# Autodesk Inventor assembly: wahacz_zewn_zlozenie
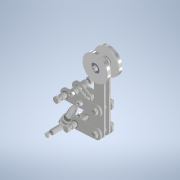
[picture p0: Inventor's stored thumbnail of the model, 180x180]
Saved by Autodesk Inventor 2020.3 (Build 243373000, 373)
## iProperties
Created: 2021-10-24
Part Number: wahacz_zewn_zlozenie
Document SubType Name: Assembly
Designer: patry
Author: patry
## Documents named in this file (26)
- C:\Users\patry\Desktop\Semestr 7\Inzynierka\Projekt inventor\Ariadna_inzynierka\Workspaces\Obszar roboczy\Obszar roboczy\Naped\Zawieszenie_v3\wahacz_zewn_zlozenie.iam
- C:\Users\patry\Desktop\Semestr 7\Inzynierka\Projekt inventor\Ariadna_inzynierka\Workspaces\Obszar roboczy\Obszar roboczy\Naped\Zawieszenie_v3\ramie_1_wahacza.ipt
- C:\Users\patry\Desktop\Semestr 7\Inzynierka\Projekt inventor\Ariadna_inzynierka\Workspaces\Obszar roboczy\Obszar roboczy\Naped\Zawieszenie_v3\ramie_2_wahacza.ipt
- C:\Users\patry\Desktop\Semestr 7\Inzynierka\Projekt inventor\Ariadna_inzynierka\Workspaces\Obszar roboczy\Obszar roboczy\Naped\Zawieszenie_v3\tuleja_TUF106040.ipt
- C:\Users\patry\Desktop\Semestr 7\Inzynierka\Projekt inventor\Ariadna_inzynierka\Workspaces\Obszar roboczy\Obszar roboczy\Naped\Sruby\M6_nut_5mm.ipt
- C:\Users\patry\Desktop\Semestr 7\Inzynierka\Projekt inventor\Ariadna_inzynierka\Workspaces\Obszar roboczy\Obszar roboczy\Naped\Amortyzator\Korpus.ipt
- C:\Users\patry\Desktop\Semestr 7\Inzynierka\Projekt inventor\Ariadna_inzynierka\Workspaces\Obszar roboczy\Obszar roboczy\Naped\Amortyzator\Tlok.ipt
- C:\Users\patry\Desktop\Semestr 7\Inzynierka\Projekt inventor\Ariadna_inzynierka\Workspaces\Obszar roboczy\Obszar roboczy\Naped\Amortyzator\Nakretka.ipt
- C:\Users\patry\Desktop\Semestr 7\Inzynierka\Projekt inventor\Ariadna_inzynierka\Workspaces\Obszar roboczy\Obszar roboczy\Naped\Sruby\M5_nut_5mm.ipt
- C:\Users\patry\Desktop\Semestr 7\Inzynierka\Projekt inventor\Ariadna_inzynierka\Workspaces\Obszar roboczy\Obszar roboczy\Naped\Sruby\M5_70_shaft.ipt
- C:\Users\patry\Desktop\Semestr 7\Inzynierka\Projekt inventor\Ariadna_inzynierka\Workspaces\Obszar roboczy\Obszar roboczy\Naped\Sruby\M3_16_shaft.ipt
- C:\Users\patry\Desktop\Semestr 7\Inzynierka\Projekt inventor\Ariadna_inzynierka\Workspaces\Obszar roboczy\Obszar roboczy\Naped\Sruby\M3_nut_2,5mm.ipt
- C:\Users\patry\Desktop\Semestr 7\Inzynierka\Projekt inventor\Ariadna_inzynierka\Workspaces\Obszar roboczy\Obszar roboczy\Naped\Zawieszenie_v3\wspornik_amortyzatora.ipt
- C:\Users\patry\Desktop\Semestr 7\Inzynierka\Projekt inventor\Ariadna_inzynierka\Workspaces\Obszar roboczy\Obszar roboczy\Naped\Sruby\M6_40_shaft.ipt
- C:\Users\patry\Desktop\Semestr 7\Inzynierka\Projekt inventor\Ariadna_inzynierka\Workspaces\Obszar roboczy\Obszar roboczy\Naped\Sruby\tuleja_M6_M10_7.ipt
- C:\Users\patry\Desktop\Semestr 7\Inzynierka\Projekt inventor\Ariadna_inzynierka\Workspaces\Obszar roboczy\Obszar roboczy\Naped\Sruby\M6_1,25_pad.ipt
- C:\Users\patry\Desktop\Semestr 7\Inzynierka\Projekt inventor\Ariadna_inzynierka\Workspaces\Obszar roboczy\Obszar roboczy\Naped\Sruby\M6_70_shaft.ipt
- C:\Users\patry\Desktop\Semestr 7\Inzynierka\Projekt inventor\Ariadna_inzynierka\Workspaces\Obszar roboczy\Obszar roboczy\Naped\Sruby\M5_40_shaft.ipt
- M5_shaft.ipt
- C:\Users\patry\Desktop\Semestr 7\Inzynierka\Projekt inventor\Ariadna_inzynierka\Workspaces\Obszar roboczy\Obszar roboczy\Naped\Sruby\tuleja_M5_M9_20.ipt
- C:\Users\patry\Desktop\Semestr 7\Inzynierka\Projekt inventor\Ariadna_inzynierka\Workspaces\Obszar roboczy\Obszar roboczy\Naped\Sruby\tuleja_M5_M9_25.ipt
- C:\Users\patry\Desktop\Semestr 7\Inzynierka\Projekt inventor\Ariadna_inzynierka\Workspaces\Obszar roboczy\Obszar roboczy\Naped\Sruby\tuleja_M5_M9_4,5.ipt
- C:\Users\patry\Desktop\Semestr 7\Inzynierka\Projekt inventor\Ariadna_inzynierka\Workspaces\Obszar roboczy\Obszar roboczy\Naped\Zawieszenie_v3\glowny_wahacz_zewn.ipt
- C:\Users\patry\Desktop\Semestr 7\Inzynierka\Projekt inventor\Ariadna_inzynierka\Workspaces\Obszar roboczy\Obszar roboczy\Naped\Sruby\tuleja_M6_M10_8,5.ipt
- C:\Users\patry\Desktop\Semestr 7\Inzynierka\Projekt inventor\Ariadna_inzynierka\Workspaces\Obszar roboczy\Obszar roboczy\Naped\Sruby\tuleja_M6_M10_13,5.ipt
- C:\Users\patry\Desktop\Semestr 7\Inzynierka\Projekt inventor\Ariadna_inzynierka\Workspaces\Obszar roboczy\Obszar roboczy\Naped\Zawieszenie_v3\independent_wheel_pair.iam
## Components (65 placed, 24 different names)
1. ramie_1_wahacza:1 — Zestawiające:7, Zestawiające:8, Kątowe:4, Zestawiające:108, Zestawiające:109, Zestawiające:110, Równoległe:6, Zestawiające:114, Zestawiające:158, Równoległe:11, Zestawiające:159, Równoległe:12, Zestawiające:161, Zestawiające:163, Zestawiające:175, Zestawiające:179, Zestawiające:203, Zestawiające:204
2. ramie_2_wahacza:1 — Zestawiające:1, Zestawiające:2, Kątowe:1, Zestawiające:118, Zestawiające:206, Zestawiające:207
3. tuleja_TUF106040:1 — Zestawiające:1, Zestawiające:2, Kątowe:1, Zestawiające:93, Zestawiające:200
4. tuleja_TUF106040:2 — Zestawiające:205, Zestawiające:206, Zestawiające:207, Zestawiające:217
5. tuleja_TUF106040:3 — Zestawiające:202, Zestawiające:203, Zestawiające:204, Zestawiające:219
6. tuleja_TUF106040:4 — Zestawiające:7, Zestawiające:8, Kątowe:4, Zestawiające:111, Zestawiające:132
7. tuleja_TUF106040:5 — Zestawiające:89, Zestawiające:201, Zestawiające:216
8. tuleja_TUF106040:6 — Zestawiające:88, Zestawiające:90, Zestawiające:189, Zestawiające:198
9. ramie_2_wahacza:2 — Równoległe:7, Zestawiające:120, Zestawiające:209, Zestawiające:210
10. tuleja_TUF106040:7 — Zestawiające:93, Zestawiające:112, Zestawiające:140
11. tuleja_TUF106040:8 — Zestawiające:208, Zestawiające:209, Zestawiające:210, Zestawiające:212
12. M6_nut_5mm:2 — Zestawiające:113, Zestawiające:114
13. Korpus:1 — Walcowe:1, Zestawiające:83, Równoległe:4, Zestawiające:87, Zestawiające:169, Zestawiające:171
14. Tlok:1 — Walcowe:1, Zestawiające:102, Zestawiające:103
15. Nakretka:1
16. M5_nut_5mm:1 — Zestawiające:84, Zestawiające:86, Zestawiające:87, Równoległe:9, Równoległe:10
17. M5_70_shaft:1 — Zestawiające:83, Równoległe:4, Zestawiające:84, Zestawiające:85, Zestawiające:143, Równoległe:8, Zestawiające:168, Zestawiające:170
18. ramie_1_wahacza:3 — Zestawiające:88, Zestawiające:89, Zestawiające:90, Zestawiające:116, Zestawiające:165, Zestawiające:167, Zestawiające:173, Zestawiające:177, Zestawiające:201
19. M5_nut_5mm:2 — Zestawiające:85, Zestawiające:86
20. M3_16_shaft:1 — Zestawiające:97, Równoległe:5, Zestawiające:98, Zestawiające:100, Zestawiające:102
21. M3_nut_2,5mm:1 — Zestawiające:98, Zestawiające:99
22. M3_nut_2,5mm:2 — Zestawiające:100, Zestawiające:101
23. wspornik_amortyzatora:1 — Zestawiające:94, Zestawiające:95, Zestawiające:96, Równoległe:5, Zestawiające:99, Zestawiające:108, Zestawiające:109, Zestawiające:110
24. wspornik_amortyzatora:2 — Zestawiające:94, Zestawiające:95, Zestawiające:96, Zestawiające:97, Zestawiające:101, Zestawiające:103
25. M6_40_shaft:1 — Zestawiające:111, Równoległe:6, Zestawiające:113, Zestawiające:115, Zestawiające:121, Zestawiające:127, Zestawiające:131, Zestawiające:182, Zestawiające:186, Zestawiające:189
26. M6_40_shaft:2 — Zestawiające:112, Równoległe:7, Zestawiające:117, Zestawiające:119, Zestawiające:123, Zestawiające:135, Zestawiające:139, Zestawiające:180, Zestawiające:185
27. M6_nut_5mm:11 — Zestawiające:115, Zestawiające:116
28. M6_nut_5mm:12 — Zestawiające:117, Zestawiające:118
29. M6_nut_5mm:13 — Zestawiające:119, Zestawiające:120
30. tuleja_M6_M10_7:1 — Zestawiające:121, Zestawiające:196
31. tuleja_M6_M10_7:2 — Zestawiające:123, Zestawiające:181
32. M6_1,25_pad:1 — Zestawiające:125, Zestawiające:126, Zestawiające:127, Zestawiające:197
33. M6_1,25_pad:2 — Zestawiające:125, Zestawiające:126, Zestawiające:198
34. M6_1,25_pad:3 — Zestawiające:131, Zestawiające:132
35. M6_1,25_pad:4 — Zestawiające:194
36. M6_1,25_pad:5 — Zestawiające:135, Zestawiające:199
37. M6_1,25_pad:6 — Zestawiające:200
38. M6_1,25_pad:7 — Zestawiające:139, Zestawiające:140
39. M6_1,25_pad:8 — Zestawiające:195
40. M6_70_shaft:1 — Zestawiające:143, Zestawiające:149, Zestawiające:205, Zestawiające:208, Zestawiające:211, Zestawiające:213
41. M6_70_shaft:2 — Równoległe:8, Zestawiające:144, Zestawiające:145, Zestawiające:202, Zestawiające:215, Zestawiające:218
42. M6_nut_5mm:14 — Zestawiające:144, Zestawiające:146
43. M6_nut_5mm:15 — Zestawiające:145, Zestawiające:146, Równoległe:9
44. M6_nut_5mm:16 — Zestawiające:148, Zestawiające:149
45. M6_nut_5mm:17 — Zestawiające:148, Równoległe:10
46. M5_shaft:1 — Zestawiające:158, Równoległe:11, Zestawiające:162, Zestawiające:164, Zestawiające:172, Zestawiające:174
47. M5_shaft:2 — Zestawiające:159, Równoległe:12, Zestawiające:160, Zestawiające:166, Zestawiające:176, Zestawiające:178
48. M5_nut_5mm:3 — Zestawiające:160, Zestawiające:161
49. M5_nut_5mm:4 — Zestawiające:162, Zestawiające:163
50. M5_nut_5mm:5 — Zestawiające:164, Zestawiające:165
51. M5_nut_5mm:6 — Zestawiające:166, Zestawiające:167
52. tuleja_M5_M9_20:1 — Zestawiające:168, Zestawiające:169
53. tuleja_M5_M9_25:1 — Zestawiające:170, Zestawiające:171
54. tuleja_M5_M9_4,5:1 — Zestawiające:172, Zestawiające:173
55. tuleja_M5_M9_4,5:2 — Zestawiające:174, Zestawiające:175
56. tuleja_M5_M9_4,5:3 — Zestawiające:176, Zestawiające:177
57. tuleja_M5_M9_4,5:4 — Zestawiające:178, Zestawiające:179
58. glowny_wahacz_zewn:1 — Zestawiające:180, Zestawiające:181, Zestawiające:182, Zestawiające:196, Zestawiające:197, Zestawiające:199
59. glowny_wahacz_zewn:2 — Zestawiające:185, Zestawiające:186, Zestawiające:194, Zestawiające:195, Zestawiające:221, Zestawiające:222, Zestawiające:223
60. tuleja_M6_M10_8,5:1 — Zestawiające:211, Zestawiające:212
61. tuleja_M6_M10_13,5:1 — Zestawiające:213, Zestawiające:217
62. tuleja_M6_M10_13,5:2 — Zestawiające:215, Zestawiające:216
63. tuleja_M6_M10_8,5:2 — Zestawiające:218, Zestawiające:219
64. independent_wheel_pair:1 [sub-assembly] — Zestawiające:221, Zestawiające:222
65. tuleja_M6_M10_7:3 — Zestawiające:223
## Relationships (135: Mate 121, Flush 9, Angle 4, CylindricalJoint 1)
- Zestawiające:1 [Mate]: ramie_2_wahacza:1 ↔ tuleja_TUF106040:1
- Zestawiające:2 [Mate]: ramie_2_wahacza:1 ↔ tuleja_TUF106040:1
- Kątowe:1 [Angle] (0 deg): ramie_2_wahacza:1 ↔ tuleja_TUF106040:1
- Zestawiające:7 [Mate]: ramie_1_wahacza:1 ↔ tuleja_TUF106040:4
- Zestawiające:8 [Mate]: ramie_1_wahacza:1 ↔ tuleja_TUF106040:4
- Kątowe:4 [Angle] (0 deg): ramie_1_wahacza:1 ↔ tuleja_TUF106040:4
- [Mate]: ramie_2_wahacza:2 ↔ tuleja_TUF106040:7
- [Mate]: ramie_2_wahacza:2 ↔ tuleja_TUF106040:7
- [Angle] (0 deg): ramie_2_wahacza:2 ↔ tuleja_TUF106040:7
- [Mate]: Korpus:1 ↔ Tlok:1
- [Angle] (0 deg): Korpus:1 ↔ Tlok:1
- [Mate]: Korpus:1 ↔ Nakretka:1
- [Mate] (5 mm): Korpus:1 ↔ Nakretka:1
- Walcowe:1 [CylindricalJoint]: Korpus:1 ↔ Tlok:1
- Zestawiające:83 [Mate]: Korpus:1 ↔ M5_70_shaft:1
- Równoległe:4 [Flush] (-30 mm): Korpus:1 ↔ M5_70_shaft:1
- Zestawiające:84 [Mate]: M5_nut_5mm:1 ↔ M5_70_shaft:1
- Zestawiające:85 [Mate]: M5_70_shaft:1 ↔ M5_nut_5mm:2
- Zestawiające:86 [Mate] (60 mm): M5_nut_5mm:1 ↔ M5_nut_5mm:2
- Zestawiające:87 [Mate] (30 mm): Korpus:1 ↔ M5_nut_5mm:1
- Zestawiające:88 [Mate]: tuleja_TUF106040:6 ↔ ramie_1_wahacza:3
- Zestawiające:89 [Mate]: tuleja_TUF106040:5 ↔ ramie_1_wahacza:3
- Zestawiające:90 [Mate]: tuleja_TUF106040:6 ↔ ramie_1_wahacza:3
- Zestawiające:93 [Mate]: tuleja_TUF106040:1 ↔ tuleja_TUF106040:7
- Zestawiające:94 [Mate]: wspornik_amortyzatora:1 ↔ wspornik_amortyzatora:2
- Zestawiające:95 [Mate]: wspornik_amortyzatora:1 ↔ wspornik_amortyzatora:2
- Zestawiające:96 [Mate] (5 mm): wspornik_amortyzatora:1 ↔ wspornik_amortyzatora:2
- Zestawiające:97 [Mate]: M3_16_shaft:1 ↔ wspornik_amortyzatora:2
- Równoległe:5 [Flush] (-2.5 mm): M3_16_shaft:1 ↔ wspornik_amortyzatora:1
- Zestawiające:98 [Mate]: M3_16_shaft:1 ↔ M3_nut_2,5mm:1
- Zestawiające:99 [Mate]: M3_nut_2,5mm:1 ↔ wspornik_amortyzatora:1
- Zestawiające:100 [Mate]: M3_16_shaft:1 ↔ M3_nut_2,5mm:2
- Zestawiające:101 [Mate]: M3_nut_2,5mm:2 ↔ wspornik_amortyzatora:2
- Zestawiające:102 [Mate]: Tlok:1 ↔ M3_16_shaft:1
- Zestawiające:103 [Mate]: Tlok:1 ↔ wspornik_amortyzatora:2
- Zestawiające:108 [Mate]: ramie_1_wahacza:1 ↔ wspornik_amortyzatora:1
- Zestawiające:109 [Mate]: ramie_1_wahacza:1 ↔ wspornik_amortyzatora:1
- Zestawiające:110 [Mate] (4.5 mm): ramie_1_wahacza:1 ↔ wspornik_amortyzatora:1
- Zestawiające:111 [Mate]: tuleja_TUF106040:4 ↔ M6_40_shaft:1
- Równoległe:6 [Flush] (7 mm): ramie_1_wahacza:1 ↔ M6_40_shaft:1
- Zestawiające:112 [Mate]: tuleja_TUF106040:7 ↔ M6_40_shaft:2
- Równoległe:7 [Flush] (7 mm): ramie_2_wahacza:2 ↔ M6_40_shaft:2
- Zestawiające:113 [Mate]: M6_nut_5mm:2 ↔ M6_40_shaft:1
- Zestawiające:114 [Mate]: ramie_1_wahacza:1 ↔ M6_nut_5mm:2
- Zestawiające:115 [Mate]: M6_40_shaft:1 ↔ M6_nut_5mm:11
- Zestawiające:116 [Mate]: ramie_1_wahacza:3 ↔ M6_nut_5mm:11
- Zestawiające:117 [Mate]: M6_40_shaft:2 ↔ M6_nut_5mm:12
- Zestawiające:118 [Mate]: ramie_2_wahacza:1 ↔ M6_nut_5mm:12
- Zestawiające:119 [Mate]: M6_40_shaft:2 ↔ M6_nut_5mm:13
- Zestawiające:120 [Mate]: ramie_2_wahacza:2 ↔ M6_nut_5mm:13
- Zestawiające:121 [Mate]: M6_40_shaft:1 ↔ tuleja_M6_M10_7:1
- Zestawiające:123 [Mate]: M6_40_shaft:2 ↔ tuleja_M6_M10_7:2
- Zestawiające:125 [Mate]: M6_1,25_pad:1 ↔ M6_1,25_pad:2
- Zestawiające:126 [Mate]: M6_1,25_pad:1 ↔ M6_1,25_pad:2
- Zestawiające:127 [Mate]: M6_40_shaft:1 ↔ M6_1,25_pad:1
- [Mate]: M6_1,25_pad:3 ↔ M6_1,25_pad:4
- [Mate]: M6_1,25_pad:3 ↔ M6_1,25_pad:4
- Zestawiające:131 [Mate]: M6_40_shaft:1 ↔ M6_1,25_pad:3
- Zestawiające:132 [Mate]: tuleja_TUF106040:4 ↔ M6_1,25_pad:3
- [Mate]: M6_1,25_pad:5 ↔ M6_1,25_pad:6
- [Mate]: M6_1,25_pad:5 ↔ M6_1,25_pad:6
- Zestawiające:135 [Mate]: M6_40_shaft:2 ↔ M6_1,25_pad:5
- [Mate]: M6_1,25_pad:7 ↔ M6_1,25_pad:8
- [Mate]: M6_1,25_pad:7 ↔ M6_1,25_pad:8
- Zestawiające:139 [Mate]: M6_40_shaft:2 ↔ M6_1,25_pad:7
- Zestawiające:140 [Mate]: tuleja_TUF106040:7 ↔ M6_1,25_pad:7
- Zestawiające:143 [Mate]: M5_70_shaft:1 ↔ M6_70_shaft:1
- Równoległe:8 [Flush]: M5_70_shaft:1 ↔ M6_70_shaft:2
- Zestawiające:144 [Mate]: M6_70_shaft:2 ↔ M6_nut_5mm:14
- Zestawiające:145 [Mate]: M6_70_shaft:2 ↔ M6_nut_5mm:15
- Zestawiające:146 [Mate] (60 mm): M6_nut_5mm:14 ↔ M6_nut_5mm:15
- Równoległe:9 [Flush]: M5_nut_5mm:1 ↔ M6_nut_5mm:15
- [Mate] (60 mm): M6_nut_5mm:16 ↔ M6_nut_5mm:17
- Zestawiające:148 [Mate]: M6_nut_5mm:16 ↔ M6_nut_5mm:17
- Zestawiające:149 [Mate]: M6_70_shaft:1 ↔ M6_nut_5mm:16
- Równoległe:10 [Flush]: M5_nut_5mm:1 ↔ M6_nut_5mm:17
- Zestawiające:158 [Mate]: ramie_1_wahacza:1 ↔ M5_shaft:1
- Równoległe:11 [Flush] (7 mm): ramie_1_wahacza:1 ↔ M5_shaft:1
- Zestawiające:159 [Mate]: ramie_1_wahacza:1 ↔ M5_shaft:2
- Równoległe:12 [Flush] (7 mm): ramie_1_wahacza:1 ↔ M5_shaft:2
- Zestawiające:160 [Mate]: M5_shaft:2 ↔ M5_nut_5mm:3
- Zestawiające:161 [Mate]: ramie_1_wahacza:1 ↔ M5_nut_5mm:3
- Zestawiające:162 [Mate]: M5_shaft:1 ↔ M5_nut_5mm:4
- Zestawiające:163 [Mate]: ramie_1_wahacza:1 ↔ M5_nut_5mm:4
- Zestawiające:164 [Mate]: M5_shaft:1 ↔ M5_nut_5mm:5
- Zestawiające:165 [Mate]: ramie_1_wahacza:3 ↔ M5_nut_5mm:5
- Zestawiające:166 [Mate]: M5_shaft:2 ↔ M5_nut_5mm:6
- Zestawiające:167 [Mate]: ramie_1_wahacza:3 ↔ M5_nut_5mm:6
- Zestawiające:168 [Mate]: M5_70_shaft:1 ↔ tuleja_M5_M9_20:1
- Zestawiające:169 [Mate]: Korpus:1 ↔ tuleja_M5_M9_20:1
- Zestawiające:170 [Mate]: M5_70_shaft:1 ↔ tuleja_M5_M9_25:1
- Zestawiające:171 [Mate]: Korpus:1 ↔ tuleja_M5_M9_25:1
- Zestawiające:172 [Mate]: M5_shaft:1 ↔ tuleja_M5_M9_4,5:1
- Zestawiające:173 [Mate]: ramie_1_wahacza:3 ↔ tuleja_M5_M9_4,5:1
- Zestawiające:174 [Mate]: M5_shaft:1 ↔ tuleja_M5_M9_4,5:2
- Zestawiające:175 [Mate]: ramie_1_wahacza:1 ↔ tuleja_M5_M9_4,5:2
- Zestawiające:176 [Mate]: M5_shaft:2 ↔ tuleja_M5_M9_4,5:3
- Zestawiające:177 [Mate]: ramie_1_wahacza:3 ↔ tuleja_M5_M9_4,5:3
- Zestawiające:178 [Mate]: M5_shaft:2 ↔ tuleja_M5_M9_4,5:4
- Zestawiające:179 [Mate]: ramie_1_wahacza:1 ↔ tuleja_M5_M9_4,5:4
- Zestawiające:180 [Mate]: M6_40_shaft:2 ↔ glowny_wahacz_zewn:1
- Zestawiające:181 [Mate]: tuleja_M6_M10_7:2 ↔ glowny_wahacz_zewn:1
- Zestawiające:182 [Mate]: M6_40_shaft:1 ↔ glowny_wahacz_zewn:1
- Zestawiające:185 [Mate]: M6_40_shaft:2 ↔ glowny_wahacz_zewn:2
- Zestawiające:186 [Mate]: M6_40_shaft:1 ↔ glowny_wahacz_zewn:2
- Zestawiające:189 [Mate]: tuleja_TUF106040:6 ↔ M6_40_shaft:1
- Zestawiające:194 [Mate]: M6_1,25_pad:4 ↔ glowny_wahacz_zewn:2
- Zestawiające:195 [Mate]: M6_1,25_pad:8 ↔ glowny_wahacz_zewn:2
- Zestawiające:196 [Mate]: tuleja_M6_M10_7:1 ↔ glowny_wahacz_zewn:1
- Zestawiające:197 [Mate]: M6_1,25_pad:1 ↔ glowny_wahacz_zewn:1
- Zestawiające:198 [Mate]: tuleja_TUF106040:6 ↔ M6_1,25_pad:2
- Zestawiające:199 [Mate]: M6_1,25_pad:5 ↔ glowny_wahacz_zewn:1
- Zestawiające:200 [Mate]: tuleja_TUF106040:1 ↔ M6_1,25_pad:6
- Zestawiające:201 [Mate]: tuleja_TUF106040:5 ↔ ramie_1_wahacza:3
- Zestawiające:202 [Mate]: tuleja_TUF106040:3 ↔ M6_70_shaft:2
- Zestawiające:203 [Mate]: ramie_1_wahacza:1 ↔ tuleja_TUF106040:3
- Zestawiające:204 [Mate]: ramie_1_wahacza:1 ↔ tuleja_TUF106040:3
- Zestawiające:205 [Mate]: tuleja_TUF106040:2 ↔ M6_70_shaft:1
- Zestawiające:206 [Mate]: ramie_2_wahacza:1 ↔ tuleja_TUF106040:2
- Zestawiające:207 [Mate]: ramie_2_wahacza:1 ↔ tuleja_TUF106040:2
- Zestawiające:208 [Mate]: tuleja_TUF106040:8 ↔ M6_70_shaft:1
- Zestawiające:209 [Mate]: ramie_2_wahacza:2 ↔ tuleja_TUF106040:8
- Zestawiające:210 [Mate]: ramie_2_wahacza:2 ↔ tuleja_TUF106040:8
- Zestawiające:211 [Mate]: M6_70_shaft:1 ↔ tuleja_M6_M10_8,5:1
- Zestawiające:212 [Mate]: tuleja_TUF106040:8 ↔ tuleja_M6_M10_8,5:1
- Zestawiające:213 [Mate]: M6_70_shaft:1 ↔ tuleja_M6_M10_13,5:1
- Zestawiające:215 [Mate]: M6_70_shaft:2 ↔ tuleja_M6_M10_13,5:2
- Zestawiające:216 [Mate]: tuleja_TUF106040:5 ↔ tuleja_M6_M10_13,5:2
- Zestawiające:217 [Mate]: tuleja_TUF106040:2 ↔ tuleja_M6_M10_13,5:1
- Zestawiające:218 [Mate]: M6_70_shaft:2 ↔ tuleja_M6_M10_8,5:2
- Zestawiające:219 [Mate]: tuleja_TUF106040:3 ↔ tuleja_M6_M10_8,5:2
- [Mate]: independent_wheel_pair:1 ↔ tuleja_M6_M10_7:3
- Zestawiające:221 [Mate]: glowny_wahacz_zewn:2 ↔ independent_wheel_pair:1
- Zestawiające:222 [Mate]: glowny_wahacz_zewn:2 ↔ independent_wheel_pair:1
- Zestawiające:223 [Mate]: glowny_wahacz_zewn:2 ↔ tuleja_M6_M10_7:3
## Named parameters: d41_d4 = 0 deg, d43_d0 = 0 mm, d44_d1 = 0 mm, d83_d6 = -2 mm, d84_d7 = -2 mm, d85_d8 = -13 mm, d86_d0 = 0 mm, d87_d1 = 0 deg, d88_d3 = 0 mm, d89_d4 = 5 mm, d90_d5 = 0 deg, d158_d154 = 0 mm, d159_d155 = 0 mm, d162_d154 = 0 mm, d163_d155 = 0 mm, d166_d154 = 0 mm, d167_d155 = 0 mm, d178_d176 = 60 mm
